# Autodesk Inventor assembly: Pi 4 Minimalistic Case - Basic
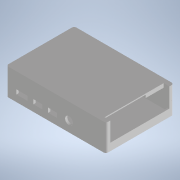
[picture p0: Inventor's stored thumbnail of the model, 180x180]
Saved by Autodesk Inventor 2020 (Build 240168000, 168)
## iProperties
Created: 2021-01-01
Part Number: Pi 4 Minimalistic Case - Basic
Document SubType Name: Assembly
Designer: frost
Author: frost
## Documents named in this file (3)
- C:\Users\frost\OneDrive\Desktop\Pi 4 Minimalistic Case - Basic.iam
- C:\Users\frost\OneDrive\Desktop\Pi 4 Case - Back Panel.ipt
- C:\Users\frost\OneDrive\Desktop\Pi 4 Case  - Upper Panel.ipt
## Components (2 placed, 2 different names)
1. Pi 4 Case - Back Panel:1 — Mate:1, Flush:1, Flush:2
2. Pi 4 Case  - Upper Panel:1 — Mate:1, Flush:1, Flush:2
## Relationships (3: Flush 2, Mate 1)
- Mate:1: Pi 4 Case - Back Panel:1 ↔ Pi 4 Case  - Upper Panel:1
- Flush:1: Pi 4 Case - Back Panel:1 ↔ Pi 4 Case  - Upper Panel:1
- Flush:2: Pi 4 Case - Back Panel:1 ↔ Pi 4 Case  - Upper Panel:1
